# Autodesk Inventor assembly: Assembly1
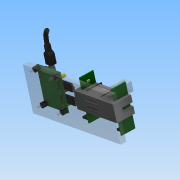
[picture p0: Inventor's stored thumbnail of the model, 180x180]
Saved by Autodesk Inventor 2016 (Build 200138000, 138)
## iProperties
Created: 2015-08-01
Part Number: Assembly1
Document SubType Name: Assembly
Designer: Openlab
Author: Openlab
## Documents named in this file (9)
- D:\Alexey\HS-Spectrophotometer\parts\Spirulina\Assembly1.iam
- D:\Alexey\HS-Spectrophotometer\parts\Spirulina\Spirulina_base.ipt
- D:\Alexey\HS-Spectrophotometer\parts\Spirulina\Spirulina_core.ipt
- D:\Alexey\HS-Spectrophotometer\parts\Common\Microcontroller_board_Nano_square.iam
- D:\Alexey\HS-Spectrophotometer\parts\Common\Support_washer.ipt
- D:\Alexey\HS-Spectrophotometer\parts\Test\LED_board.ipt
- D:\Alexey\HS-Spectrophotometer\parts\Test\Sensor_board.ipt
- D:\Alexey\HS-Spectrophotometer\parts\Test\Distance_test_adaptor_circle_2mm.ipt
- D:\Alexey\HS-Spectrophotometer\parts\Common\Cuvette.ipt
## Components (12 placed, 8 different names)
1. Spirulina_base:1 — Mate:1, Mate:2, Mate:3, Mate:4, Mate:5, Mate:6, Mate:7, Mate:8, Mate:9, Flush:5, Flush:6
2. Spirulina_core:1 — Mate:1, Mate:13, Mate:14, Mate:15, Mate:16, Mate:17, Mate:18, Flush:3, Flush:4, Mate:19, Mate:20, Mate:21, Flush:5, Flush:6
3. Microcontroller_board_Nano_square:1 [sub-assembly] — Mate:10, Mate:11, Mate:12
4. Support_washer:1 — Mate:2, Mate:6
5. Support_washer:2 — Mate:3, Mate:7, Mate:11
6. Support_washer:3 — Mate:4, Mate:8, Mate:10, Mate:12
7. Support_washer:4 — Mate:5, Mate:9
8. LED_board:1 — Mate:15, Mate:16
9. Sensor_board:1 — Mate:13, Mate:14
10. Distance_test_adaptor_circle_2mm:1 — Mate:17, Flush:3
11. Distance_test_adaptor_circle_2mm:2 — Mate:18, Flush:4
12. Cuvette:1 — Mate:19, Mate:20, Mate:21
## Relationships (25: Mate 21, Flush 4)
- Mate:1: Spirulina_base:1 ↔ Spirulina_core:1
- Mate:2: Spirulina_base:1 ↔ Support_washer:1
- Mate:3: Spirulina_base:1 ↔ Support_washer:2
- Mate:4: Spirulina_base:1 ↔ Support_washer:3
- Mate:5: Spirulina_base:1 ↔ Support_washer:4
- Mate:6: Spirulina_base:1 ↔ Support_washer:1
- Mate:7: Spirulina_base:1 ↔ Support_washer:2
- Mate:8: Spirulina_base:1 ↔ Support_washer:3
- Mate:9: Spirulina_base:1 ↔ Support_washer:4
- Mate:10: Microcontroller_board_Nano_square:1 ↔ Support_washer:3
- Mate:11: Microcontroller_board_Nano_square:1 ↔ Support_washer:2
- Mate:12: Microcontroller_board_Nano_square:1 ↔ Support_washer:3
- Mate:13: Spirulina_core:1 ↔ Sensor_board:1
- Mate:14: Spirulina_core:1 ↔ Sensor_board:1
- Mate:15: Spirulina_core:1 ↔ LED_board:1
- Mate:16: Spirulina_core:1 ↔ LED_board:1
- Mate:17: Spirulina_core:1 ↔ Distance_test_adaptor_circle_2mm:1
- Mate:18: Spirulina_core:1 ↔ Distance_test_adaptor_circle_2mm:2
- Flush:3: Spirulina_core:1 ↔ Distance_test_adaptor_circle_2mm:1
- Flush:4: Spirulina_core:1 ↔ Distance_test_adaptor_circle_2mm:2
- Mate:19: Spirulina_core:1 ↔ Cuvette:1
- Mate:20: Spirulina_core:1 ↔ Cuvette:1
- Mate:21: Spirulina_core:1 ↔ Cuvette:1
- Flush:5 (10 mm): Spirulina_base:1 ↔ Spirulina_core:1
- Flush:6 (20 mm): Spirulina_base:1 ↔ Spirulina_core:1
